# Autodesk Inventor assembly: motorDriveWheelAssembly
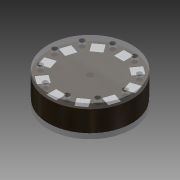
[picture p0: Inventor's stored thumbnail of the model, 180x180]
Saved by Autodesk Inventor 2013 (Build 170138000, 138)
## iProperties
Created: 2013-01-21
Part Number: motorDriveWheelAssembly
Document SubType Name: Assembly
Designer: Nano
Author: Nano
## Documents named in this file (6)
- C:\Users\Nano\Documents\InventorByron\InventorMasterProject\gyroPhone01\motorDriveWheelAssembly.iam
- C:\Users\Nano\Documents\InventorByron\InventorMasterProject\gyroPhone01\motorBodyAndShaftMassive01.ipt
- C:\Users\Nano\Documents\InventorByron\InventorMasterProject\gyroPhone01\driveWheel01.ipt
- C:\Users\Nano\Documents\InventorByron\InventorMasterProject\gyroPhone01\magnet1_4x1_4x1_2.ipt
- C:\Users\Nano\Documents\InventorByron\InventorMasterProject\gyroPhone01\topPlate.ipt
- C:\Users\Nano\Documents\InventorByron\InventorMasterProject\gyroPhone01\basePlate.ipt
## Components (14 placed, 5 different names)
1. motorBodyAndShaftMassive01:1 — Flush:1
2. driveWheel01:1 — Flush:1, Mate:1, Mate:2, Flush:2, Flush:3, Flush:4, Flush:5, Flush:6
3. topPlate:1 — Flush:3, Flush:4
4. basePlate:1 — Flush:5, Flush:6
5. magnet1_4x1_4x1_2:1 — Mate:1, Mate:2, Flush:2
6. magnet1_4x1_4x1_2:2
7. magnet1_4x1_4x1_2:3
8. magnet1_4x1_4x1_2:4
9. magnet1_4x1_4x1_2:5
10. magnet1_4x1_4x1_2:6
11. magnet1_4x1_4x1_2:7
12. magnet1_4x1_4x1_2:8
13. magnet1_4x1_4x1_2:9
14. magnet1_4x1_4x1_2:10
## Component patterns: (10 elements, first: magnet1_4x1_4x1_2:1)
## Relationships (8: Flush 6, Mate 2)
- Flush:1: motorBodyAndShaftMassive01:1 ↔ driveWheel01:1
- Mate:1: driveWheel01:1 ↔ magnet1_4x1_4x1_2:1
- Mate:2: driveWheel01:1 ↔ magnet1_4x1_4x1_2:1
- Flush:2: driveWheel01:1 ↔ magnet1_4x1_4x1_2:1
- Flush:3: driveWheel01:1 ↔ topPlate:1
- Flush:4: driveWheel01:1 ↔ topPlate:1
- Flush:5: driveWheel01:1 ↔ basePlate:1
- Flush:6: driveWheel01:1 ↔ basePlate:1
